# Autodesk Inventor assembly: Major_Finger_assembly_1
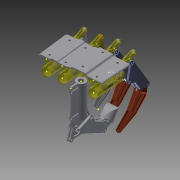
[picture p0: Inventor's stored thumbnail of the model, 180x180]
Saved by Autodesk Inventor 2015 (Build 190159000, 159)
## iProperties
Created: 2016-10-25
Part Number: Major_Finger_assembly_1
Document SubType Name: Assembly
Designer: Neelotpal Nag
Author: Neelotpal Nag
## Documents named in this file (6)
- D:\NEEL BACKUP\DISA 2016\Fingers 1\Major_Finger_assembly_1.iam
- D:\NEEL BACKUP\DISA 2016\Fingers 1\Finger_New_Support_base_Screwing.ipt
- D:\NEEL BACKUP\DISA 2016\Fingers 1\Index+Middle\Index_Finger_assembly_1.iam
- D:\NEEL BACKUP\DISA 2016\Fingers 1\Ring\Ring_Finger_assembly_1.iam
- D:\NEEL BACKUP\DISA 2016\Fingers 1\Pinky\Pinky_Assembly_01.iam
- D:\NEEL BACKUP\DISA 2016\Fingers 1\Thumb\Thumb_assembly_1.iam
## Components (6 placed, 5 different names)
1. Finger_New_Support_base_Screwing:1 — Mate:1, Mate:2, Mate:3, Mate:4, Mate:5, Mate:6, Mate:7, Mate:8, Mate:9, Mate:10, Mate:11, Mate:12
2. Index_Finger_assembly_1:1 [sub-assembly] — Mate:1, Mate:2, Mate:3, Angle:1, Angle:2
3. Index_Finger_assembly_1:2 [sub-assembly] — Mate:4, Mate:5, Mate:6
4. Ring_Finger_assembly_1:1 [sub-assembly] — Mate:7, Mate:8, Mate:9
5. Pinky_Assembly_01:1 [sub-assembly] — Mate:10, Mate:11, Mate:12
6. Thumb_assembly_1:1 [sub-assembly] — Angle:1, Angle:2
## Relationships (14: Mate 12, Angle 2)
- Mate:1: Finger_New_Support_base_Screwing:1 ↔ Index_Finger_assembly_1:1
- Mate:2: Finger_New_Support_base_Screwing:1 ↔ Index_Finger_assembly_1:1
- Mate:3: Finger_New_Support_base_Screwing:1 ↔ Index_Finger_assembly_1:1
- Mate:4: Finger_New_Support_base_Screwing:1 ↔ Index_Finger_assembly_1:2
- Mate:5: Finger_New_Support_base_Screwing:1 ↔ Index_Finger_assembly_1:2
- Mate:6: Finger_New_Support_base_Screwing:1 ↔ Index_Finger_assembly_1:2
- Mate:7: Finger_New_Support_base_Screwing:1 ↔ Ring_Finger_assembly_1:1
- Mate:8: Finger_New_Support_base_Screwing:1 ↔ Ring_Finger_assembly_1:1
- Mate:9: Finger_New_Support_base_Screwing:1 ↔ Ring_Finger_assembly_1:1
- Mate:10: Finger_New_Support_base_Screwing:1 ↔ Pinky_Assembly_01:1
- Mate:11: Finger_New_Support_base_Screwing:1 ↔ Pinky_Assembly_01:1
- Mate:12: Finger_New_Support_base_Screwing:1 ↔ Pinky_Assembly_01:1
- Angle:1 (90 deg): Index_Finger_assembly_1:1 ↔ Thumb_assembly_1:1
- Angle:2 (0 deg): Index_Finger_assembly_1:1 ↔ Thumb_assembly_1:1
